# Autodesk Inventor assembly: PowerpolePairWContacts
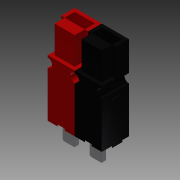
[picture p0: Inventor's stored thumbnail of the model, 180x180]
Saved by Autodesk Inventor 2014 SP1 (Build 180222100, 222)
## iProperties
Created: 2016-03-18
Part Number: PowerpolePairWContacts
Document SubType Name: Assembly
Designer: Tyler
Author: Tyler
## Documents named in this file (3)
- C:\Users\Tyler\Documents\powerpolebreakout\Cad\PowerpolePairWContacts.iam
- C:\Users\Tyler\Documents\powerpolebreakout\Cad\PowerPole45.ipt
- C:\Users\Tyler\Documents\powerpolebreakout\Cad\Powerpole45APCBStraight.ipt
## Components (4 placed, 2 different names)
1. PowerPole45:1 — Flush:1, Mate:1, Flush:2, Mate:2, Mate:3, Mate:4
2. PowerPole45:2 — Flush:1, Mate:1, Flush:2, Mate:5, Mate:6, Mate:7
3. Powerpole45APCBStraight:1 — Mate:5, Mate:6, Mate:7
4. Powerpole45APCBStraight:2 — Mate:2, Mate:3, Mate:4
## Relationships (9: Mate 7, Flush 2)
- Flush:1: PowerPole45:1 ↔ PowerPole45:2
- Mate:1: PowerPole45:1 ↔ PowerPole45:2
- Flush:2: PowerPole45:1 ↔ PowerPole45:2
- Mate:2: PowerPole45:1 ↔ Powerpole45APCBStraight:2
- Mate:3: PowerPole45:1 ↔ Powerpole45APCBStraight:2
- Mate:4: PowerPole45:1 ↔ Powerpole45APCBStraight:2
- Mate:5: PowerPole45:2 ↔ Powerpole45APCBStraight:1
- Mate:6: PowerPole45:2 ↔ Powerpole45APCBStraight:1
- Mate:7: PowerPole45:2 ↔ Powerpole45APCBStraight:1
